# Autodesk Inventor assembly: rudder
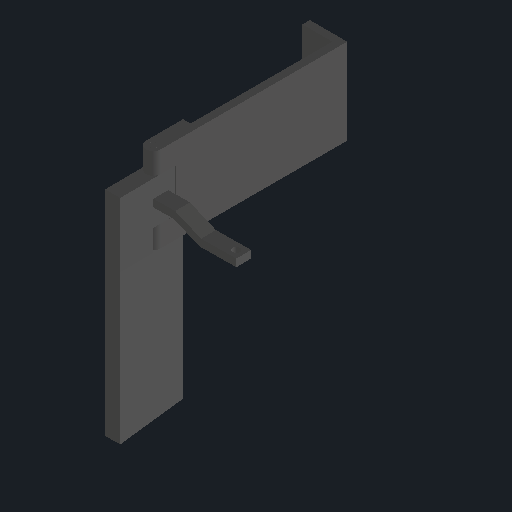
[picture p0: Inventor's stored thumbnail of the model, 512x512]
Saved by Autodesk Inventor 2024 (Build 280153000, 153)
## iProperties
Created: 2022-03-30
Part Number: rudder
Document SubType Name: Assembly
Designer: kardo
Mass: 5.74394 g
Surface Area: 60.4549 cm^2
Volume: 5.74394 cm^3
Density: 1 g/cm^3
Author: kardo
## Documents named in this file (3)
- D:\Computer Aided Design\hydroplane_plan_2_refactor\model\shape\frame\hardware\rudder.iam
- D:\Computer Aided Design\hydroplane_plan_2_refactor\model\shape\frame\hardware\rudder_base.ipt
- D:\Computer Aided Design\hydroplane_plan_2_refactor\model\shape\frame\hardware\rudder_fin.ipt
## Components (2 placed, 2 different names)
1. rudder_base:1 — Mate:1, Cylindrical:1
2. rudder_fin:1 — Mate:1, Cylindrical:1
## Relationships (2: Mate 1, CylindricalJoint 1)
- Mate:1: rudder_base:1 ↔ rudder_fin:1
- Cylindrical:1: rudder_base:1 ↔ rudder_fin:1
